# Autodesk Inventor assembly: Wheel mount
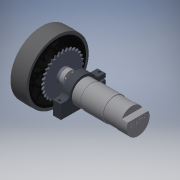
[picture p0: Inventor's stored thumbnail of the model, 180x180]
Saved by Autodesk Inventor 2016 (Build 200138000, 138)
## iProperties
Created: 2015-11-11
Part Number: Wheel mount
Document SubType Name: Assembly
Designer: Julia
Author: Julia
## Documents named in this file (6)
- C:\Users\Julia\Documents\FTC CAD Parts\Wheel mount.iam
- C:\Users\Julia\Documents\FTC CAD Parts\Andy Mark\am-2648_4inWheel8mmHub.ipt
- C:\Users\Julia\Documents\FTC CAD Parts\Andy Mark\am-2964NeveRest.ipt
- C:\Users\Julia\Documents\FTC CAD Parts\Tetrix_Kit_FTC\tetrix_739171_sprk_25_32t_2013.ipt
- C:\Users\Julia\Documents\FTC CAD Parts\Tetrix_Kit_FTC\tetrix_739079_collar_2012.ipt
- C:\Users\Julia\Documents\FTC CAD Parts\Tetrix_Kit_FTC\tetrix_739089_2012.ipt
## Components (6 placed, 5 different names)
1. am-2648_4inWheel8mmHub:1 — Mate:4
2. am-2964NeveRest:1 — Mate:1, Mate:2, Mate:3, Mate:4, Mate:5
3. tetrix_739171_sprk_25_32t_2013:1 — Mate:2
4. tetrix_739079_collar_2012:1 — Mate:3
5. tetrix_739079_collar_2012:2 — Mate:1
6. tetrix_739089_2012:1 — Mate:5
## Relationships (5: Mate 5)
- Mate:1: am-2964NeveRest:1 ↔ tetrix_739079_collar_2012:2
- Mate:2: am-2964NeveRest:1 ↔ tetrix_739171_sprk_25_32t_2013:1
- Mate:3: am-2964NeveRest:1 ↔ tetrix_739079_collar_2012:1
- Mate:4: am-2648_4inWheel8mmHub:1 ↔ am-2964NeveRest:1
- Mate:5: am-2964NeveRest:1 ↔ tetrix_739089_2012:1
